# Autodesk Inventor assembly: RobotArm_v3
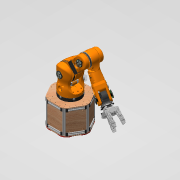
[picture p0: Inventor's stored thumbnail of the model, 180x180]
Saved by Autodesk Inventor 2016 (Build 200138000, 138)
## iProperties
Created: 2015-03-01
Part Number: RobotArm_v3
Document SubType Name: Assembly
Designer: 4ndreas
Author: 4ndreas
## Documents named in this file (9)
- C:\Users\4ndreas\Documents\Inventor\RobotARM v2\v3\RobotArm_v3.iam
- C:\Users\4ndreas\Documents\Inventor\RobotARM v2\v3\Shoulder.iam
- C:\Users\4ndreas\Documents\Inventor\RobotARM v2\v3\SE_Spacer.ipt
- C:\Users\4ndreas\Documents\Inventor\RobotARM v2\v3\Ellbow.iam
- C:\Users\4ndreas\Documents\Inventor\RobotARM v2\v3\wrist.iam
- C:\Users\4ndreas\Documents\Inventor\RobotARM v2\v3\Gripper_Mount.iam
- C:\Users\4ndreas\Documents\Inventor\Gripper\openHand\3_finger_gripper.iam
- C:\Users\4ndreas\Documents\Inventor\RobotARM v2\v3\RotaryBase.iam
- C:\Users\4ndreas\Documents\Inventor\RobotARM v2\v3\SimpleBase_v1.iam
## Components (8 placed, 8 different names)
1. SimpleBase_v1:1 [sub-assembly] — Passend:1, Passend:17, Passend:18, Passend:19
2. RotaryBase:1 [sub-assembly] — Passend:15, Passend:16, Passend:17, Passend:18, Passend:19
3. Shoulder:1 [sub-assembly] — Passend:2, Fluchtend:1, Fluchtend:2, Passend:15, Passend:16
4. SE_Spacer:1 — Passend:2, Fluchtend:1, Fluchtend:2, Passend:3, Passend:4, Passend:5
5. Ellbow:2 [sub-assembly] — Passend:3, Passend:4, Passend:5, Passend:6, Passend:7
6. wrist:1 [sub-assembly] — Passend:6, Passend:7, Passend:8, Passend:9
7. Gripper_Mount:1 [sub-assembly] — Passend:8, Passend:9, Passend:13, Passend:14, Fluchtend:4
8. 3_finger_gripper:1 [sub-assembly] — Passend:13, Passend:14, Fluchtend:4
## Relationships (19: Mate 16, Flush 3)
- Passend:1 [Mate]: SimpleBase_v1:1
- Passend:2 [Mate]: Shoulder:1 ↔ SE_Spacer:1
- Fluchtend:1 [Flush]: Shoulder:1 ↔ SE_Spacer:1
- Fluchtend:2 [Flush]: Shoulder:1 ↔ SE_Spacer:1
- Passend:3 [Mate]: SE_Spacer:1 ↔ Ellbow:2
- Passend:4 [Mate]: SE_Spacer:1 ↔ Ellbow:2
- Passend:5 [Mate]: SE_Spacer:1 ↔ Ellbow:2
- Passend:6 [Mate]: Ellbow:2 ↔ wrist:1
- Passend:7 [Mate] (2 mm): Ellbow:2 ↔ wrist:1
- Passend:8 [Mate]: wrist:1 ↔ Gripper_Mount:1
- Passend:9 [Mate]: wrist:1 ↔ Gripper_Mount:1
- Passend:13 [Mate]: Gripper_Mount:1 ↔ 3_finger_gripper:1
- Passend:14 [Mate]: Gripper_Mount:1 ↔ 3_finger_gripper:1
- Fluchtend:4 [Flush]: Gripper_Mount:1 ↔ 3_finger_gripper:1
- Passend:15 [Mate]: RotaryBase:1 ↔ Shoulder:1
- Passend:16 [Mate]: RotaryBase:1 ↔ Shoulder:1
- Passend:17 [Mate]: SimpleBase_v1:1 ↔ RotaryBase:1
- Passend:18 [Mate]: SimpleBase_v1:1 ↔ RotaryBase:1
- Passend:19 [Mate]: SimpleBase_v1:1 ↔ RotaryBase:1
